# Autodesk Inventor assembly: Shoulder_support_assembly
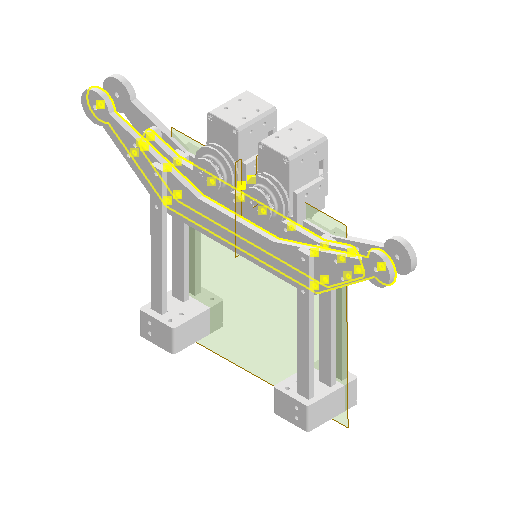
[picture p0: Inventor's stored thumbnail of the model, 512x512]
Saved by Autodesk Inventor 2022 (Build 260153000, 153)
## iProperties
Created: 2022-08-23
Part Number: Shoulder_support_assembly
Document SubType Name: Assembly
Designer: dell
Mass: 215.1 g
Surface Area: 1120.32 cm^2
Volume: 215.1 cm^3
Author: dell
## Documents named in this file (9)
- D:\xxxx\Uni\Part IV\MECHENG_700\Part_IV_project_CAD\Bird_skeleton_prototypes\Wing_drone_V1\Bird_wing_V2\Wing_shoulder\Shoulder_support_assembly.iam
- D:\xxxx\Uni\Part IV\MECHENG_700\Part_IV_project_CAD\Bird_skeleton_prototypes\Wing_drone_V1\Bird_wing_V2\Wing_shoulder\Vertical_bar.ipt
- D:\xxxx\Uni\Part IV\MECHENG_700\Part_IV_project_CAD\Bird_skeleton_prototypes\Wing_drone_V1\Bird_wing_V2\Wing_shoulder\Bar_connection_assembly.iam
- D:\xxxx\Uni\Part IV\MECHENG_700\Part_IV_project_CAD\Bird_skeleton_prototypes\Wing_drone_V1\Bird_wing_V2\Wing_shoulder\Horizontal_bar_V2.ipt
- D:\xxxx\Uni\Part IV\MECHENG_700\Part_IV_project_CAD\Bird_skeleton_prototypes\Wing_drone_V1\Bird_wing_V2\Motor_pulley_assembly.iam
- D:\xxxx\Uni\Part IV\MECHENG_700\Part_IV_project_CAD\Bird_skeleton_prototypes\Wing_drone_V1\Bird_wing_V2\Wing_shoulder\Horizontal_bar_support_V2.ipt
- D:\xxxx\Uni\Part IV\MECHENG_700\Part_IV_project_CAD\Bird_skeleton_prototypes\Wing_drone_V1\Bird_wing_V2\Wing_shoulder\Horizontal_bar_spacer.ipt
- D:\xxxx\Uni\Part IV\MECHENG_700\Part_IV_project_CAD\Bird_skeleton_prototypes\Wing_drone_V1\Bird_wing_V2\Wing_shoulder\Horizontal_bar_p2_V2.ipt
- D:\xxxx\Uni\Part IV\MECHENG_700\Part_IV_project_CAD\Bird_skeleton_prototypes\Wing_drone_V1\Bird_wing_V2\Wing_shoulder\Horizontal_bar_spacer_small.ipt
## Components (17 placed, 8 different names)
1. Vertical_bar:1 — Flush:1, Flush:4, Mate:5, Symmetry:1, Mate:12
2. Vertical_bar:2 — Flush:1, Flush:4, Mate:9, Mate:10, Flush:8, Mate:12, Mate:13, Mate:17
3. Vertical_bar:3 — Flush:2, Flush:3, Symmetry:1, Mate:7, Mate:8, Flush:7, Mate:15, Mate:18
4. Vertical_bar:4 — Flush:2, Flush:3, Mate:5, Mate:16, Mate:26, Mate:27
5. Bar_connection_assembly:1 [sub-assembly] — Mate:9, Mate:10, Flush:8, Mate:48, Mate:49
6. Bar_connection_assembly:2 [sub-assembly] — Mate:7, Mate:8, Flush:7, Mate:50, Mate:51
7. Horizontal_bar_V2:1 — Mate:13, Mate:15, Mate:16, Mate:17, Mate:18, Mate:19, Mate:20, Mate:21, Mate:23, Mate:24, Mate:25, Mate:28, Mate:30
8. Motor_pulley_assembly:3 [sub-assembly] — Mate:19, Mate:20, Mate:21, Mate:22
9. Motor_pulley_assembly:4 [sub-assembly] — Mate:23, Mate:24, Mate:25
10. Horizontal_bar_support_V2:2 — Mate:26, Mate:27, Mate:29, Mate:31, Mate:41, Mate:42, Mate:43
11. Horizontal_bar_spacer:4 — Mate:30, Mate:31
12. Horizontal_bar_spacer:5 — Mate:28, Mate:29
13. Horizontal_bar_p2_V2:1 — Mate:41, Mate:42, Mate:43, Mate:44, Mate:45, Mate:46, Mate:47
14. Horizontal_bar_spacer_small:1 — Mate:44, Mate:45
15. Horizontal_bar_spacer_small:2 — Mate:46, Mate:47
16. Vertical_bar:5 — Mate:48, Mate:49
17. Vertical_bar:6 — Mate:50, Mate:51
## Relationships (42: Mate 35, Flush 6, Symmetry 1)
- Flush:1: Vertical_bar:1 ↔ Vertical_bar:2
- Flush:2: Vertical_bar:3 ↔ Vertical_bar:4
- Flush:3: Vertical_bar:3 ↔ Vertical_bar:4
- Flush:4: Vertical_bar:1 ↔ Vertical_bar:2
- Mate:5 (120 mm): Vertical_bar:1 ↔ Vertical_bar:4
- Symmetry:1: Vertical_bar:1 ↔ Vertical_bar:3
- Mate:7: Vertical_bar:3 ↔ Bar_connection_assembly:2
- Mate:8: Vertical_bar:3 ↔ Bar_connection_assembly:2
- Flush:7: Vertical_bar:3 ↔ Bar_connection_assembly:2
- Mate:9: Vertical_bar:2 ↔ Bar_connection_assembly:1
- Mate:10: Vertical_bar:2 ↔ Bar_connection_assembly:1
- Flush:8: Vertical_bar:2 ↔ Bar_connection_assembly:1
- Mate:12 (5 mm): Vertical_bar:1 ↔ Vertical_bar:2
- Mate:13: Vertical_bar:2 ↔ Horizontal_bar_V2:1
- Mate:15: Vertical_bar:3 ↔ Horizontal_bar_V2:1
- Mate:16: Vertical_bar:4 ↔ Horizontal_bar_V2:1
- Mate:17: Vertical_bar:2 ↔ Horizontal_bar_V2:1
- Mate:18: Vertical_bar:3 ↔ Horizontal_bar_V2:1
- Mate:19: Horizontal_bar_V2:1 ↔ Motor_pulley_assembly:3
- Mate:20: Horizontal_bar_V2:1 ↔ Motor_pulley_assembly:3
- Mate:21: Horizontal_bar_V2:1 ↔ Motor_pulley_assembly:3
- Mate:22: Motor_pulley_assembly:3
- Mate:23: Horizontal_bar_V2:1 ↔ Motor_pulley_assembly:4
- Mate:24: Horizontal_bar_V2:1 ↔ Motor_pulley_assembly:4
- Mate:25: Horizontal_bar_V2:1 ↔ Motor_pulley_assembly:4
- Mate:26: Vertical_bar:4 ↔ Horizontal_bar_support_V2:2
- Mate:27: Vertical_bar:4 ↔ Horizontal_bar_support_V2:2
- Mate:28: Horizontal_bar_V2:1 ↔ Horizontal_bar_spacer:5
- Mate:29: Horizontal_bar_support_V2:2 ↔ Horizontal_bar_spacer:5
- Mate:30: Horizontal_bar_V2:1 ↔ Horizontal_bar_spacer:4
- Mate:31: Horizontal_bar_support_V2:2 ↔ Horizontal_bar_spacer:4
- Mate:41 (4.2 mm): Horizontal_bar_support_V2:2 ↔ Horizontal_bar_p2_V2:1
- Mate:42: Horizontal_bar_support_V2:2 ↔ Horizontal_bar_p2_V2:1
- Mate:43: Horizontal_bar_support_V2:2 ↔ Horizontal_bar_p2_V2:1
- Mate:44: Horizontal_bar_p2_V2:1 ↔ Horizontal_bar_spacer_small:1
- Mate:45: Horizontal_bar_p2_V2:1 ↔ Horizontal_bar_spacer_small:1
- Mate:46: Horizontal_bar_p2_V2:1 ↔ Horizontal_bar_spacer_small:2
- Mate:47: Horizontal_bar_p2_V2:1 ↔ Horizontal_bar_spacer_small:2
- Mate:48: Bar_connection_assembly:1 ↔ Vertical_bar:5
- Mate:49 (0.1 mm): Bar_connection_assembly:1 ↔ Vertical_bar:5
- Mate:50: Bar_connection_assembly:2 ↔ Vertical_bar:6
- Mate:51 (0.1 mm): Bar_connection_assembly:2 ↔ Vertical_bar:6
